# Autodesk Inventor assembly: Assembly4
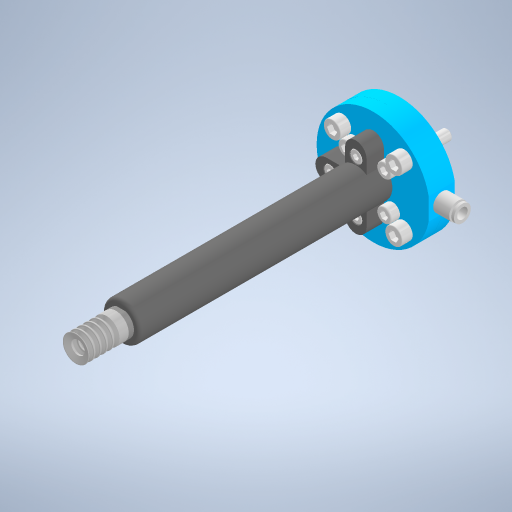
[picture p0: Inventor's stored thumbnail of the model, 512x512]
Saved by Autodesk Inventor 2023 (Build 270158000, 158)
## iProperties
Created: 2022-05-19
Part Number: Assembly4
Document SubType Name: Assembly
Designer: romanp
Author: romanp
## Documents named in this file (10)
- C:\Users\romanp\Downloads\SMC_EE_ZP2-TB15ZJS6-AL12-06\Pack_and_Go\Assembly_SMC_EE.iam
- C:\Users\romanp\Downloads\SMC_EE_ZP2-TB15ZJS6-AL12-06\Pack_and_Go\M4x20.ipt
- C:\Users\romanp\Downloads\SMC_EE_ZP2-TB15ZJS6-AL12-06\Pack_and_Go\M4_nut.ipt
- C:\Users\romanp\Downloads\SMC_EE_ZP2-TB15ZJS6-AL12-06\Pack_and_Go\ZP2-TB15ZJS6-AL12-06.ipt
- C:\Users\romanp\Downloads\SMC_EE_ZP2-TB15ZJS6-AL12-06\Pack_and_Go\KQ2H06-00A.ipt
- C:\Users\romanp\Downloads\SMC_EE_ZP2-TB15ZJS6-AL12-06\Pack_and_Go\M5x25.ipt
- C:\Users\romanp\Downloads\SMC_EE_ZP2-TB15ZJS6-AL12-06\Pack_and_Go\M6x25.ipt
- C:\Users\romanp\Downloads\SMC_EE_ZP2-TB15ZJS6-AL12-06\Pack_and_Go\Part_Top_a_Blue.ipt
- C:\Users\romanp\Downloads\SMC_EE_ZP2-TB15ZJS6-AL12-06\Pack_and_Go\Part_Top_b_Blue.ipt
- C:\Users\romanp\Downloads\SMC_EE_ZP2-TB15ZJS6-AL12-06\Pack_and_Go\Part_Bottom_Black.ipt
## Components (19 placed, 9 different names)
1. M4x20:1
2. ZP2-TB15ZJS6-AL12-06:1
3. M4x20:2
4. M4x20:3
5. M4_nut:3
6. M4_nut:4
7. M4_nut:5
8. KQ2H06-00A:1
9. M6x25:5 — Insert:15
10. M5x25:5 — Insert:16
11. Part_Top_a_Blue — Insert:14
12. Part_Top_b_Blue — Insert:14, Insert:15, Insert:16, Insert:17, Insert:18, Insert:19, Insert:20, Insert:21, Insert:22, Insert:23
13. M6x25:6 — Insert:18
14. M5x25:6 — Insert:17
15. M6x25:7 — Insert:19
16. M6x25:8 — Insert:20
17. M5x25:7 — Insert:21
18. M5x25:8 — Insert:22
19. Part_Bottom_Black — Insert:23
## Relationships (10: Insert 10)
- Insert:14: Part_Top_a_Blue ↔ Part_Top_b_Blue
- Insert:15: M6x25:5 ↔ Part_Top_b_Blue
- Insert:16: M5x25:5 ↔ Part_Top_b_Blue
- Insert:17: Part_Top_b_Blue ↔ M5x25:6
- Insert:18: Part_Top_b_Blue ↔ M6x25:6
- Insert:19: Part_Top_b_Blue ↔ M6x25:7
- Insert:20: Part_Top_b_Blue ↔ M6x25:8
- Insert:21: Part_Top_b_Blue ↔ M5x25:7
- Insert:22: Part_Top_b_Blue ↔ M5x25:8
- Insert:23: Part_Top_b_Blue ↔ Part_Bottom_Black
